# Autodesk Inventor assembly: P1704_E002
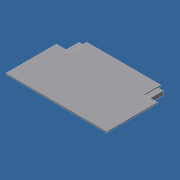
[picture p0: Inventor's stored thumbnail of the model, 180x180]
Saved by Autodesk Inventor 2019 (Build 230136000, 136)
## iProperties
Created: 2019-05-03
Part Number: P1704_E002
Project: Nom Projet
Description: Ens. Nom Ensemble
Document SubType Name: Assembly
Designer: Joan.MAILLARD
Author: Joan.MAILLARD
## Documents named in this file (3)
- P:\projet_manette\manette\06_Dessins\P1704_E002.iam
- P:\projet_manette\manette\06_Dessins\P1704_008_pcb.ipt
- P:\projet_manette\manette\06_Dessins\P1704_009_slider.ipt
## Components (3 placed, 2 different names)
1. P1704_008_pcb:1 — Glissière:1, Glissière:2
2. P1704_009_slider:1 — Glissière:1
3. P1704_009_slider:2 — Glissière:2
## Relationships (2: TranslationJoint 2)
- Glissière:1 [TranslationJoint]: P1704_008_pcb:1 ↔ P1704_009_slider:1
- Glissière:2 [TranslationJoint]: P1704_008_pcb:1 ↔ P1704_009_slider:2
